# Autodesk Inventor assembly: ppt_platform
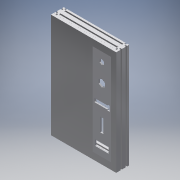
[picture p0: Inventor's stored thumbnail of the model, 180x180]
Saved by Autodesk Inventor 2016 (Build 200138000, 138)
## iProperties
Created: 2016-01-21
Part Number: ppt_platform
Document SubType Name: Assembly
Designer: Fred
Author: Fred
## Documents named in this file (7)
- E:\DOCUMENTS\ROBOCUP-AT-WORK\MODELS\ARENA\elements\platform\ppt\inventor\ppt_platform.iam
- E:\DOCUMENTS\ROBOCUP-AT-WORK\MODELS\ARENA\elements\platform\service_area\inventor\platform_800x500x99_assembly.iam
- E:\documents\robocup-at-work\models\ppt_cavities\horizontal\S40_40_B_AND_G_HORIZONTAL.IPT
- E:\documents\robocup-at-work\models\ppt_cavities\horizontal\F20_20_B_AND_G_HORIZONTAL.IPT
- E:\documents\robocup-at-work\models\ppt_cavities\horizontal\M20_100_HORIZONTAL.IPT
- E:\documents\robocup-at-work\models\ppt_cavities\horizontal\M30_HORIZONTAL.IPT
- E:\documents\robocup-at-work\models\ppt_cavities\horizontal\M20_HORIZONTAL.IPT
## Components (6 placed, 6 different names)
1. platform_800x500x99_assembly:1 [sub-assembly] — Mate:1, Mate:2, Mate:3, Mate:4, Mate:6, Mate:7, Mate:8, Mate:9, Mate:10, Mate:11, Mate:12, Mate:13
2. S40_40_B_AND_G_HORIZONTAL:1 — Mate:1, Mate:2, Mate:3, Mate:5
3. F20_20_B_AND_G_HORIZONTAL:1 — Mate:4, Mate:5, Mate:6, Mate:15
4. M20_100_HORIZONTAL:1 — Mate:7, Mate:8, Mate:15
5. M30_HORIZONTAL:1 — Mate:9, Mate:10, Mate:14
6. M20_HORIZONTAL:1 — Mate:11, Mate:12, Mate:13, Mate:14
## Relationships (15: Mate 15)
- Mate:1: platform_800x500x99_assembly:1 ↔ S40_40_B_AND_G_HORIZONTAL:1
- Mate:2: platform_800x500x99_assembly:1 ↔ S40_40_B_AND_G_HORIZONTAL:1
- Mate:3: platform_800x500x99_assembly:1 ↔ S40_40_B_AND_G_HORIZONTAL:1
- Mate:4: platform_800x500x99_assembly:1 ↔ F20_20_B_AND_G_HORIZONTAL:1
- Mate:5: S40_40_B_AND_G_HORIZONTAL:1 ↔ F20_20_B_AND_G_HORIZONTAL:1
- Mate:6: platform_800x500x99_assembly:1 ↔ F20_20_B_AND_G_HORIZONTAL:1
- Mate:7: platform_800x500x99_assembly:1 ↔ M20_100_HORIZONTAL:1
- Mate:8: platform_800x500x99_assembly:1 ↔ M20_100_HORIZONTAL:1
- Mate:9: platform_800x500x99_assembly:1 ↔ M30_HORIZONTAL:1
- Mate:10: platform_800x500x99_assembly:1 ↔ M30_HORIZONTAL:1
- Mate:11: platform_800x500x99_assembly:1 ↔ M20_HORIZONTAL:1
- Mate:12: platform_800x500x99_assembly:1 ↔ M20_HORIZONTAL:1
- Mate:13: platform_800x500x99_assembly:1 ↔ M20_HORIZONTAL:1
- Mate:14: M30_HORIZONTAL:1 ↔ M20_HORIZONTAL:1
- Mate:15: F20_20_B_AND_G_HORIZONTAL:1 ↔ M20_100_HORIZONTAL:1
